# Autodesk Inventor assembly: AM Shifter Output Shaft subassembly
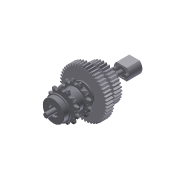
[picture p0: Inventor's stored thumbnail of the model, 180x180]
Saved by Autodesk Inventor 2011 (Build 150239000, 239)
## iProperties
Created: 2012-06-03
Part Number: AM Shifter Output Shaft subassembly
Document SubType Name: Assembly
Designer: Nemo
Author: Nemo
## Documents named in this file (13)
- H:\Nemo\Documents\Robotics\COTS Parts\Gearboxes\Shafts\AM Shifter Output Shaft subassembly.iam
- H:\Nemo\Documents\Robotics\COTS Parts\Gearboxes\Shafts\AM Shifter Output Hex Shaft.ipt
- H:\Nemo\Documents\Robotics\COTS Parts\Gearboxes\Bearings\Bearing FR6zz.ipt
- H:\Nemo\Documents\Robotics\COTS Parts\Gearboxes\Bearings\Bearing FR8zz.ipt
- H:\Nemo\Documents\Robotics\COTS Parts\Gearboxes\Bearings\Bearing FR6.ipt
- H:\Nemo\Documents\Robotics\COTS Parts\Gearboxes\Gears\Gear 20dp 875dog 35T.ipt
- H:\Nemo\Documents\Robotics\COTS Parts\Gearboxes\Shifters\Dog Gear.ipt
- H:\Nemo\Documents\Robotics\COTS Parts\Gearboxes\Shifters\Roll Pin 925x100.ipt
- H:\Nemo\Documents\Robotics\COTS Parts\Gearboxes\Shifters\Shift Block subassembly.iam
- H:\Nemo\Documents\Robotics\COTS Parts\Sprockets\35 sprocket 12T 500key.ipt
- H:\Nemo\Documents\Robotics\COTS Parts\Gearboxes\Gears\Gear 20dp 1125dog 48T.ipt
- H:\Nemo\Documents\Robotics\COTS Parts\Gearboxes\Bearings\Bearing R8.ipt
- H:\Nemo\Documents\Robotics\COTS Parts\Gearboxes\Spacers\Washer - shifter spacing.ipt
## Components (19 placed, 12 different names)
1. AM Shifter Output Hex Shaft:1 — Mate:1, Insert:4, Mate:3, Angle:1, Mate:4, Mate:8, Angle:3, Mate:9
2. Bearing FR6zz:1 — Insert:3, Mate:2
3. Bearing FR8zz:1 — Mate:1, Mate:2, Insert:7
4. Bearing FR6:1 — Insert:2, Insert:3, Insert:4
5. Gear 35T dog shift:1 — Insert:2
6. Dog Gear:1 — Mate:3, Angle:1, Insert:5
7. Roll Pin 925x100:1 — Insert:5, Mate:5
8. Shift Block subassembly:1 [sub-assembly] — Mate:4, Mate:5
9. 35 sprocket 12T 500key:1 — Mate:6, Mate:7, Angle:2, Insert:13
10. 35 sprocket 12T 500key:2 — Mate:6, Mate:7, Angle:2, Mate:8, Angle:3, Insert:10
11. Gear 48T dog shift:1 — Insert:6
12. Bearing R8:1 — Insert:6, Mate:9, Mate:10
13. Washer - shifter spacing:1 — Insert:12, Insert:14
14. Washer - shifter spacing:2 — Insert:11, Insert:12
15. Washer - shifter spacing:3 — Insert:10, Insert:11
16. Washer - shifter spacing:4 — Insert:9, Insert:13
17. Washer - shifter spacing:5 — Insert:8, Insert:9
18. Washer - shifter spacing:6 — Insert:7, Insert:8
19. Washer - shifter spacing:7 — Insert:14, Mate:10
## Relationships (26: Insert 13, Mate 10, Angle 3)
- Mate:1: AM Shifter Output Hex Shaft:1 ↔ Bearing FR8zz:1
- Insert:2: Bearing FR6:1 ↔ Gear 35T dog shift:1
- Insert:3: Bearing FR6zz:1 ↔ Bearing FR6:1
- Insert:4: AM Shifter Output Hex Shaft:1 ↔ Bearing FR6:1
- Mate:2 (-66.04 mm): Bearing FR6zz:1 ↔ Bearing FR8zz:1
- Mate:3: AM Shifter Output Hex Shaft:1 ↔ Dog Gear:1
- Angle:1 (0 deg): AM Shifter Output Hex Shaft:1 ↔ Dog Gear:1
- Insert:5: Dog Gear:1 ↔ Roll Pin 925x100:1
- Mate:4: AM Shifter Output Hex Shaft:1 ↔ Shift Block subassembly:1
- Mate:5: Roll Pin 925x100:1 ↔ Shift Block subassembly:1
- Mate:6: 35 sprocket 12T 500key:1 ↔ 35 sprocket 12T 500key:2
- Mate:7: 35 sprocket 12T 500key:1 ↔ 35 sprocket 12T 500key:2
- Angle:2 (0 deg): 35 sprocket 12T 500key:1 ↔ 35 sprocket 12T 500key:2
- Mate:8: AM Shifter Output Hex Shaft:1 ↔ 35 sprocket 12T 500key:2
- Angle:3 (0 deg): AM Shifter Output Hex Shaft:1 ↔ 35 sprocket 12T 500key:2
- Insert:6: Gear 48T dog shift:1 ↔ Bearing R8:1
- Mate:9: AM Shifter Output Hex Shaft:1 ↔ Bearing R8:1
- Insert:7: Bearing FR8zz:1 ↔ Washer - shifter spacing:6
- Insert:8: Washer - shifter spacing:5 ↔ Washer - shifter spacing:6
- Insert:9: Washer - shifter spacing:4 ↔ Washer - shifter spacing:5
- Insert:10: 35 sprocket 12T 500key:2 ↔ Washer - shifter spacing:3
- Insert:11: Washer - shifter spacing:2 ↔ Washer - shifter spacing:3
- Insert:12: Washer - shifter spacing:1 ↔ Washer - shifter spacing:2
- Insert:13: 35 sprocket 12T 500key:1 ↔ Washer - shifter spacing:4
- Insert:14: Washer - shifter spacing:1 ↔ Washer - shifter spacing:7
- Mate:10: Bearing R8:1 ↔ Washer - shifter spacing:7
